# Autodesk Inventor assembly: calf_left
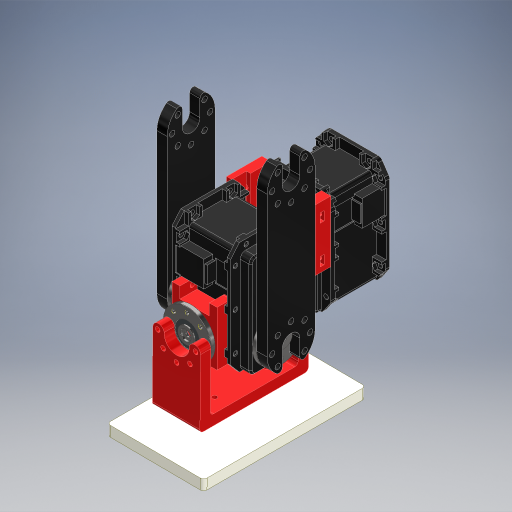
[picture p0: Inventor's stored thumbnail of the model, 512x512]
Saved by Autodesk Inventor 2024 (Build 280153000, 153)
## iProperties
Created: 2024-09-16
Part Number: calf_left
Document SubType Name: Assembly
Designer: msi
Author: msi
## Documents named in this file (13)
- C:\Users\msi\GITHUB\19th_intern_kgh_fight_robot\부품\Lower_Body\Calf\calf_left.iam
- C:\Users\msi\GITHUB\19th_intern_kgh_fight_robot\부품\Lower_Body\Calf\knee and ankle connection.ipt
- C:\Users\msi\GITHUB\19th_intern_kgh_fight_robot\부품\Lower_Body\Calf\ankle.ipt
- foot_right_64_ver2.ipt
- C:\Users\msi\GITHUB\19th_intern_kgh_fight_robot\부품\Lower_Body\Calf\front ankle connection_left.ipt
- C:\Users\msi\GITHUB\19th_intern_kgh_fight_robot\부품\Lower_Body\Calf\behind ankle connection_outside.ipt
- C:\Users\msi\GITHUB\19th_intern_kgh_fight_robot\부품\Lower_Body\Calf\behind ankle connection_inside.ipt
- C:\Users\msi\GITHUB\19th_intern_kgh_fight_robot\부품\ROBOTIS(Inventor 2024 ver.)\다이나믹셀\MX-106T+idle.ipt.iam
- C:\Users\msi\GITHUB\19th_intern_kgh_fight_robot\부품\ROBOTIS(Inventor 2024 ver.)\다이나믹셀\MX-64T.ipt
- C:\Users\msi\GITHUB\19th_intern_kgh_fight_robot\부품\ROBOTIS(Inventor 2024 ver.)\혼\64-106Horn.ipt
- C:\Users\msi\GITHUB\19th_intern_kgh_fight_robot\부품\ROBOTIS(Inventor 2024 ver.)\아이들러\64아이들러.iam
- C:\Users\msi\GITHUB\19th_intern_kgh_fight_robot\부품\Lower_Body\Calf\foot.ipt
- MX-106T+idle.ipt
## Components (12 placed, 10 different names)
1. knee and ankle connection:1 — 삽입:4, 삽입:5
2. behind ankle connection_outside:1 — 삽입:9, 삽입:10, 삽입:16, 삽입:17
3. behind ankle connection_inside:1 — 삽입:7, 삽입:8, 삽입:18, 삽입:19
4. MX-106T+idle.ipt:1 [sub-assembly] — 삽입:3, 삽입:6, 삽입:7, 삽입:8, 삽입:9, 삽입:10, 삽입:25, 삽입:26
5. MX-64T:1 — 삽입:11, 삽입:16, 삽입:17, 삽입:18, 삽입:19
6. 64-106Horn:1 — 삽입:3, 삽입:4, 삽입:5
7. knee and ankle connection:2 — 삽입:6
8. 64-106Horn:2 — 삽입:11, 삽입:12, 삽입:13
9. foot_right_64_ver2:1 — 삽입:12, 삽입:13, 삽입:23, 삽입:27, 삽입:28
10. 64아이들러:1 [sub-assembly] — 삽입:23, 삽입:24
11. front ankle connection_left:1 — 삽입:24, 삽입:25, 삽입:26
12. foot:1 — 삽입:27, 삽입:28
## Relationships (21: Insert 21)
- 삽입:3 [Insert]: MX-106T+idle.ipt:1 ↔ 64-106Horn:1
- 삽입:4 [Insert]: knee and ankle connection:1 ↔ 64-106Horn:1
- 삽입:5 [Insert]: knee and ankle connection:1 ↔ 64-106Horn:1
- 삽입:6 [Insert]: MX-106T+idle.ipt:1 ↔ knee and ankle connection:2
- 삽입:7 [Insert]: behind ankle connection_inside:1 ↔ MX-106T+idle.ipt:1
- 삽입:8 [Insert]: behind ankle connection_inside:1 ↔ MX-106T+idle.ipt:1
- 삽입:9 [Insert]: behind ankle connection_outside:1 ↔ MX-106T+idle.ipt:1
- 삽입:10 [Insert]: behind ankle connection_outside:1 ↔ MX-106T+idle.ipt:1
- 삽입:11 [Insert]: MX-64T:1 ↔ 64-106Horn:2
- 삽입:12 [Insert]: 64-106Horn:2 ↔ foot_right_64_ver2:1
- 삽입:13 [Insert]: 64-106Horn:2 ↔ foot_right_64_ver2:1
- 삽입:16 [Insert]: behind ankle connection_outside:1 ↔ MX-64T:1
- 삽입:17 [Insert]: behind ankle connection_outside:1 ↔ MX-64T:1
- 삽입:18 [Insert]: behind ankle connection_inside:1 ↔ MX-64T:1
- 삽입:19 [Insert]: behind ankle connection_inside:1 ↔ MX-64T:1
- 삽입:23 [Insert]: foot_right_64_ver2:1 ↔ 64아이들러:1
- 삽입:24 [Insert] (0.1 mm): 64아이들러:1 ↔ front ankle connection_left:1
- 삽입:25 [Insert]: MX-106T+idle.ipt:1 ↔ front ankle connection_left:1
- 삽입:26 [Insert]: MX-106T+idle.ipt:1 ↔ front ankle connection_left:1
- 삽입:27 [Insert]: foot_right_64_ver2:1 ↔ foot:1
- 삽입:28 [Insert]: foot_right_64_ver2:1 ↔ foot:1
